# Autodesk Inventor assembly: Holding Block
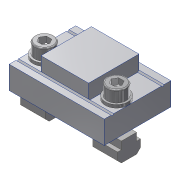
[picture p0: Inventor's stored thumbnail of the model, 180x180]
Saved by Autodesk Inventor 2016 (Build 200138000, 138)
## iProperties
Created: 2015-08-18
Part Number: Holding Block
Document SubType Name: Assembly
## Documents named in this file (5)
- E:\GitHub\CNC-Router_Accessories\Holding Block Assembly.iam
- E:\GitHub\CNC-Router_Accessories\Holding Block.ipt
- E:\GitHub\Buy-Parts\T-Nutenstein 8 - M6_St.ipt
- E:\GitHub\Standard-Parts\U-Scheibe_ISO 7089 - 6 - 140 HV_St-Vzkt.ipt
- E:\GitHub\Standard-Parts\Zyl-Schr_ISO 4762 - M6 x 20_St-Vzkt.ipt
## Components (7 placed, 4 different names)
1. Holding Block:1 — Flush:3, Mate:1, Mate:2, Mate:3, Mate:4, Mate:5
2. T-Nutenstein 8 - M6_St:1 — Flush:1, Flush:2, Flush:3, Mate:1, Mate:3, Mate:7
3. T-Nutenstein 8 - M6_St:2 — Flush:1, Flush:2, Mate:2, Mate:6
4. Zyl-Schr_ISO 4762 - M6 x 20_St-Vzkt:1 — Insert:1, Mate:6
5. U-Scheibe_ISO 7089 - 6 - 140 HV_St-Vzkt:1 — Insert:1, Mate:5
6. Zyl-Schr_ISO 4762 - M6 x 20_St-Vzkt:2 — Mate:7
7. U-Scheibe_ISO 7089 - 6 - 140 HV_St-Vzkt:2 — Mate:4
## Relationships (12: Mate 7, Flush 3, Insert 2)
- Flush:1: T-Nutenstein 8 - M6_St:1 ↔ T-Nutenstein 8 - M6_St:2
- Flush:2: T-Nutenstein 8 - M6_St:1 ↔ T-Nutenstein 8 - M6_St:2
- Flush:3 (-0.25 mm): Holding Block:1 ↔ T-Nutenstein 8 - M6_St:1
- Mate:1 (-6 mm): Holding Block:1 ↔ T-Nutenstein 8 - M6_St:1
- Mate:2 (-6 mm): Holding Block:1 ↔ T-Nutenstein 8 - M6_St:2
- Mate:3 (6 mm): Holding Block:1 ↔ T-Nutenstein 8 - M6_St:1
- Insert:1: Zyl-Schr_ISO 4762 - M6 x 20_St-Vzkt:1 ↔ U-Scheibe_ISO 7089 - 6 - 140 HV_St-Vzkt:1
- [Insert]: Zyl-Schr_ISO 4762 - M6 x 20_St-Vzkt:2 ↔ U-Scheibe_ISO 7089 - 6 - 140 HV_St-Vzkt:2
- Mate:4: Holding Block:1 ↔ U-Scheibe_ISO 7089 - 6 - 140 HV_St-Vzkt:2
- Mate:5: Holding Block:1 ↔ U-Scheibe_ISO 7089 - 6 - 140 HV_St-Vzkt:1
- Mate:6: T-Nutenstein 8 - M6_St:2 ↔ Zyl-Schr_ISO 4762 - M6 x 20_St-Vzkt:1
- Mate:7: T-Nutenstein 8 - M6_St:1 ↔ Zyl-Schr_ISO 4762 - M6 x 20_St-Vzkt:2
## Named parameters: d13_d12 = 0 mm
